# Autodesk Inventor assembly: ASY PNS 750 filter-distribution-system 1200
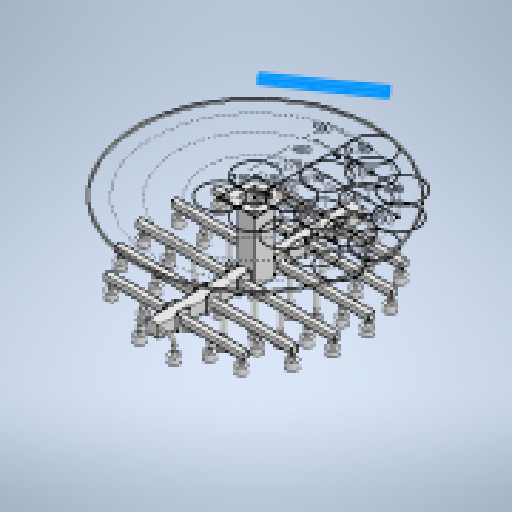
[picture p0: Inventor's stored thumbnail of the model, 512x512]
Saved by Autodesk Inventor 2025.1 (Build 291241020, 241B)
## iProperties
Created: 2025-06-24
Part Number: ASY PNS 750 filter-distribution-system 1200
Document SubType Name: Assembly
Designer: user
Author: user
## Documents named in this file (14)
- C:\Users\user\YandexDisk-badmisterfox\home pc\Inventor\PNS2-Panaevsk\filter-distribution-system\ASY PNS 750 filter-distribution-system 1200.iam
- C:\Users\user\YandexDisk-badmisterfox\home pc\Inventor\PNS2-Panaevsk\filter-distribution-system\PNS 751 DIM filter-distribution-system 1200.ipt
- C:\Users\user\YandexDisk-badmisterfox\home pc\Inventor\PNS2-Panaevsk\filter-distribution-system\PNS 754 FDS 1200 FLANGE.ipt
- C:\Users\user\YandexDisk-badmisterfox\home pc\Inventor\PNS2-Panaevsk\filter-distribution-system\PNS 752 FDS 1200 FLANGE 2.ipt
- C:\Users\user\YandexDisk-badmisterfox\home pc\Inventor\PNS2-Panaevsk\filter-distribution-system\PNS 753 FDS 1200 FLANGE 3.ipt
- C:\Users\user\YandexDisk-badmisterfox\home pc\Inventor\PNS2-Panaevsk\CC\en-US\JIS B 2312 90 (4)\JIS B 2312 90 Deg Long Elbow Stainless Steel 15A x Sch 5S.ipt
- C:\Users\user\YandexDisk-badmisterfox\home pc\Inventor\PNS2-Panaevsk\PNS dummy filter element.ipt
- C:\Users\user\YandexDisk-badmisterfox\home pc\Inventor\PNS2-Panaevsk\PNS dummy pipe nippel.ipt
- C:\Users\user\YandexDisk-badmisterfox\home pc\Inventor\PNS2-Panaevsk\filter-distribution-system\PNS 759 FDS 1200 way tube 7.ipt
- C:\Users\user\YandexDisk-badmisterfox\home pc\Inventor\PNS2-Panaevsk\filter-distribution-system\ASY PNS FDS way1.iam
- C:\Users\user\YandexDisk-badmisterfox\home pc\Inventor\PNS2-Panaevsk\filter-distribution-system\ASY PNS FDS way 2.iam
- C:\Users\user\YandexDisk-badmisterfox\home pc\Inventor\PNS2-Panaevsk\filter-distribution-system\ASY PNS FDS way3.iam
- C:\Users\user\YandexDisk-badmisterfox\home pc\Inventor\PNS2-Panaevsk\filter-distribution-system\PNS 767 FDS 1200 CUP 2.ipt
- C:\Users\user\YandexDisk-badmisterfox\home pc\Inventor\PNS2-Panaevsk\filter-distribution-system\PNS 765 FDS 1200 CUP 1.ipt
## Components (37 placed, 13 different names)
1. PNS 751 DIM filter-distribution-system 1200.ipt:1 — Mate:4, Mate:5
2. PNS 754 FDS 1200 FLANGE.ipt:1 — Mate:1, Flush:1, Flush:2
3. PNS 752 FDS 1200 FLANGE 2.ipt:1 — Rigid:1, Flush:1, Rigid:2, Mate:6, Flush:3, Flush:4
4. PNS 752 FDS 1200 FLANGE 2.ipt:2 — Rigid:1, Mate:1, Flush:2, Rigid:3
5. PNS 753 FDS 1200 FLANGE 3.ipt:1 — Rigid:2, Rigid:7, Rigid:9, Rigid:14, Rigid:15, Rigid:31, Rigid:33
6. PNS 753 FDS 1200 FLANGE 3.ipt:2 — Rigid:3, Rigid:10, Rigid:11, Rigid:12, Rigid:13, Rigid:16, Rigid:17, Rigid:29, Rigid:30, Rigid:32
7. JIS B 2312 90 Deg Long Elbow Stainless Steel 15A x Sch 5S.ipt:1 — Rigid:7, Rigid:8, Rigid:18, Rigid:19
8. PNS dummy filter element.ipt:1 — Rigid:8
9. PNS dummy pipe nippel.ipt:1 — Rigid:18
10. ASY PNS FDS way1.iam:1 [sub-assembly]
11. ASY PNS FDS way 2.iam:1 [sub-assembly]
12. ASY PNS FDS way3.iam:1 [sub-assembly]
13. ASY PNS FDS way1.iam:2 [sub-assembly] — Rigid:9
14. ASY PNS FDS way1.iam:3 [sub-assembly] — Rigid:11
15. ASY PNS FDS way1.iam:4 [sub-assembly] — Rigid:10
16. ASY PNS FDS way 2.iam:2 [sub-assembly] — Rigid:14
17. ASY PNS FDS way 2.iam:3 [sub-assembly] — Rigid:13
18. ASY PNS FDS way 2.iam:4 [sub-assembly] — Rigid:12
19. ASY PNS FDS way3.iam:2 [sub-assembly] — Rigid:15
20. ASY PNS FDS way3.iam:3 [sub-assembly] — Rigid:16
21. ASY PNS FDS way3.iam:4 [sub-assembly] — Rigid:17
22. PNS 759 FDS 1200 way tube 7.ipt:1 — Rigid:19
23. JIS B 2312 90 Deg Long Elbow Stainless Steel 15A x Sch 5S.ipt:2
24. PNS dummy filter element.ipt:2
25. PNS dummy pipe nippel.ipt:2
26. PNS 759 FDS 1200 way tube 7.ipt:2 — Rigid:31
27. JIS B 2312 90 Deg Long Elbow Stainless Steel 15A x Sch 5S.ipt:3
28. PNS dummy filter element.ipt:3
29. PNS dummy pipe nippel.ipt:3
30. PNS 759 FDS 1200 way tube 7.ipt:3 — Rigid:29
31. JIS B 2312 90 Deg Long Elbow Stainless Steel 15A x Sch 5S.ipt:4
32. PNS dummy filter element.ipt:4
33. PNS dummy pipe nippel.ipt:4
34. PNS 759 FDS 1200 way tube 7.ipt:4 — Rigid:30
35. PNS 767 FDS 1200 CUP 2.ipt:1 — Rigid:32
36. PNS 767 FDS 1200 CUP 2.ipt:2 — Rigid:33
37. PNS 765 FDS 1200 CUP 1.ipt:1 — Mate:6, Flush:3, Flush:4
## Relationships (41: WeldJoint 33, Mate 4, Flush 4)
- Rigid:1 [WeldJoint]: PNS 752 FDS 1200 FLANGE 2.ipt:1 ↔ PNS 752 FDS 1200 FLANGE 2.ipt:2
- Mate:1: PNS 754 FDS 1200 FLANGE.ipt:1 ↔ PNS 752 FDS 1200 FLANGE 2.ipt:2
- Flush:1: PNS 754 FDS 1200 FLANGE.ipt:1 ↔ PNS 752 FDS 1200 FLANGE 2.ipt:1
- Flush:2: PNS 754 FDS 1200 FLANGE.ipt:1 ↔ PNS 752 FDS 1200 FLANGE 2.ipt:2
- Mate:4: PNS 751 DIM filter-distribution-system 1200.ipt:1
- Mate:5: PNS 751 DIM filter-distribution-system 1200.ipt:1
- Rigid:2 [WeldJoint]: PNS 752 FDS 1200 FLANGE 2.ipt:1 ↔ PNS 753 FDS 1200 FLANGE 3.ipt:1
- Rigid:3 [WeldJoint]: PNS 752 FDS 1200 FLANGE 2.ipt:2 ↔ PNS 753 FDS 1200 FLANGE 3.ipt:2
- [WeldJoint] (-2 mm): PNS 753 FDS 1200 FLANGE 3.ipt:1 ↔ ASY PNS FDS way1.iam:1
- [WeldJoint] (-2 mm): PNS 753 FDS 1200 FLANGE 3.ipt:1 ↔ ASY PNS FDS way 2.iam:1
- [WeldJoint]: PNS 753 FDS 1200 FLANGE 3.ipt:1 ↔ ASY PNS FDS way3.iam:1
- Rigid:7 [WeldJoint] (-20 mm): PNS 753 FDS 1200 FLANGE 3.ipt:1 ↔ JIS B 2312 90 Deg Long Elbow Stainless Steel 15A x Sch 5S.ipt:1
- Rigid:8 [WeldJoint] (20 mm): JIS B 2312 90 Deg Long Elbow Stainless Steel 15A x Sch 5S.ipt:1 ↔ PNS dummy filter element.ipt:1
- Rigid:9 [WeldJoint]: PNS 753 FDS 1200 FLANGE 3.ipt:1 ↔ ASY PNS FDS way1.iam:2
- Rigid:10 [WeldJoint]: PNS 753 FDS 1200 FLANGE 3.ipt:2 ↔ ASY PNS FDS way1.iam:4
- Rigid:11 [WeldJoint]: PNS 753 FDS 1200 FLANGE 3.ipt:2 ↔ ASY PNS FDS way1.iam:3
- Rigid:12 [WeldJoint]: PNS 753 FDS 1200 FLANGE 3.ipt:2 ↔ ASY PNS FDS way 2.iam:4
- Rigid:13 [WeldJoint]: PNS 753 FDS 1200 FLANGE 3.ipt:2 ↔ ASY PNS FDS way 2.iam:3
- Rigid:14 [WeldJoint]: PNS 753 FDS 1200 FLANGE 3.ipt:1 ↔ ASY PNS FDS way 2.iam:2
- Rigid:15 [WeldJoint]: PNS 753 FDS 1200 FLANGE 3.ipt:1 ↔ ASY PNS FDS way3.iam:2
- Rigid:16 [WeldJoint]: PNS 753 FDS 1200 FLANGE 3.ipt:2 ↔ ASY PNS FDS way3.iam:3
- Rigid:17 [WeldJoint]: PNS 753 FDS 1200 FLANGE 3.ipt:2 ↔ ASY PNS FDS way3.iam:4
- Rigid:18 [WeldJoint]: JIS B 2312 90 Deg Long Elbow Stainless Steel 15A x Sch 5S.ipt:1 ↔ PNS dummy pipe nippel.ipt:1
- Rigid:19 [WeldJoint]: JIS B 2312 90 Deg Long Elbow Stainless Steel 15A x Sch 5S.ipt:1 ↔ PNS 759 FDS 1200 way tube 7.ipt:1
- [WeldJoint] (20 mm): JIS B 2312 90 Deg Long Elbow Stainless Steel 15A x Sch 5S.ipt:2 ↔ PNS dummy filter element.ipt:2
- [WeldJoint]: JIS B 2312 90 Deg Long Elbow Stainless Steel 15A x Sch 5S.ipt:2 ↔ PNS dummy pipe nippel.ipt:2
- [WeldJoint]: JIS B 2312 90 Deg Long Elbow Stainless Steel 15A x Sch 5S.ipt:2 ↔ PNS 759 FDS 1200 way tube 7.ipt:2
- [WeldJoint] (20 mm): JIS B 2312 90 Deg Long Elbow Stainless Steel 15A x Sch 5S.ipt:3 ↔ PNS dummy filter element.ipt:3
- [WeldJoint]: JIS B 2312 90 Deg Long Elbow Stainless Steel 15A x Sch 5S.ipt:3 ↔ PNS dummy pipe nippel.ipt:3
- [WeldJoint]: JIS B 2312 90 Deg Long Elbow Stainless Steel 15A x Sch 5S.ipt:3 ↔ PNS 759 FDS 1200 way tube 7.ipt:3
- [WeldJoint] (20 mm): JIS B 2312 90 Deg Long Elbow Stainless Steel 15A x Sch 5S.ipt:4 ↔ PNS dummy filter element.ipt:4
- [WeldJoint]: JIS B 2312 90 Deg Long Elbow Stainless Steel 15A x Sch 5S.ipt:4 ↔ PNS dummy pipe nippel.ipt:4
- [WeldJoint]: JIS B 2312 90 Deg Long Elbow Stainless Steel 15A x Sch 5S.ipt:4 ↔ PNS 759 FDS 1200 way tube 7.ipt:4
- Rigid:29 [WeldJoint]: PNS 753 FDS 1200 FLANGE 3.ipt:2 ↔ PNS 759 FDS 1200 way tube 7.ipt:3
- Rigid:30 [WeldJoint]: PNS 753 FDS 1200 FLANGE 3.ipt:2 ↔ PNS 759 FDS 1200 way tube 7.ipt:4
- Rigid:31 [WeldJoint]: PNS 753 FDS 1200 FLANGE 3.ipt:1 ↔ PNS 759 FDS 1200 way tube 7.ipt:2
- Rigid:32 [WeldJoint]: PNS 753 FDS 1200 FLANGE 3.ipt:2 ↔ PNS 767 FDS 1200 CUP 2.ipt:1
- Rigid:33 [WeldJoint]: PNS 753 FDS 1200 FLANGE 3.ipt:1 ↔ PNS 767 FDS 1200 CUP 2.ipt:2
- Mate:6: PNS 752 FDS 1200 FLANGE 2.ipt:1 ↔ PNS 765 FDS 1200 CUP 1.ipt:1
- Flush:3: PNS 752 FDS 1200 FLANGE 2.ipt:1 ↔ PNS 765 FDS 1200 CUP 1.ipt:1
- Flush:4: PNS 752 FDS 1200 FLANGE 2.ipt:1 ↔ PNS 765 FDS 1200 CUP 1.ipt:1
## Named parameters: d69_d30 = 20 mm, d70_d67 = 0 mm, d71_d68 = 0 mm, d72_d30 = 20 mm, d73_d67 = 0 mm, d74_d68 = 0 mm, d75_d30 = 20 mm, d76_d67 = 0 mm, d77_d68 = 0 mm
